# Autodesk Inventor assembly: Gear HS 60 tooth
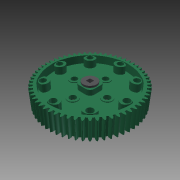
[picture p0: Inventor's stored thumbnail of the model, 180x180]
Saved by Autodesk Inventor 2015 (Build 190159000, 159)
## iProperties
Created: 2014-04-21
Part Number: Gear HS 60 tooth
Document SubType Name: Assembly
Designer: Christopher Vodney
Author: Christopher Vodney
## Documents named in this file (3)
- F:\VEX CAD Library\Motion\Gear HS 60 tooth (fixed).iam
- F:\VEX CAD Library\Motion\Insert HS Metal.ipt
- F:\VEX CAD Library\Motion\Gear HS 60 tooth.ipt
## Components (3 placed, 2 different names)
1. Gear HS 60 tooth:1 — Mate:8, Mate:9, Angle:1, Mate:10, Mate:11
2. Insert HS Metal:1 — Mate:10, Mate:11, Angle:2
3. Insert HS Metal:2 — Mate:8, Mate:9, Angle:1, Angle:2
## Relationships (6: Mate 4, Angle 2)
- Mate:8: Gear HS 60 tooth:1 ↔ Insert HS Metal:2
- Mate:9: Gear HS 60 tooth:1 ↔ Insert HS Metal:2
- Angle:1 (0 deg): Gear HS 60 tooth:1 ↔ Insert HS Metal:2
- Mate:10: Gear HS 60 tooth:1 ↔ Insert HS Metal:1
- Mate:11: Gear HS 60 tooth:1 ↔ Insert HS Metal:1
- Angle:2 (0 deg): Insert HS Metal:1 ↔ Insert HS Metal:2
